# Autodesk Inventor assembly: 途中
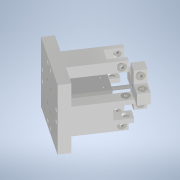
[picture p0: Inventor's stored thumbnail of the model, 180x180]
Saved by Autodesk Inventor 2021 (Build 250183000, 183)
## iProperties
Created: 2021-10-17
Part Number: 途中
Document SubType Name: Assembly
Designer: ryusei
Author: ryusei
## Documents named in this file (9)
- C:\Users\ryusei\Documents\Inventor\robot_design3\完成版\途中.iam
- C:\Users\ryusei\Documents\Inventor\robot_design3\試作品2号\部品\土台.ipt
- C:\Users\ryusei\Documents\Inventor\robot_design3\試作品2号\部品\アーム支え.ipt
- C:\Users\ryusei\Documents\Inventor\robot_design3\試作品2号\部品\シリンダ固定.ipt
- C:\Users\ryusei\Documents\Inventor\robot_design3\試作品2号\部品\MBDA6×15_シリンダコガネイ\本体.ipt
- C:\Users\ryusei\Documents\Inventor\robot_design3\試作品2号\部品\MBDA6×15_シリンダコガネイ\伸びるやつ１.ipt
- C:\Users\ryusei\Documents\Inventor\robot_design3\試作品2号\部品\MBDA6×15_シリンダコガネイ\伸びるやつ2.ipt
- C:\Users\ryusei\Documents\Inventor\robot_design3\試作品2号\部品\シリンダ先端パーツ.ipt
- C:\Users\ryusei\Documents\Inventor\robot_design3\試作品2号\部品\MF63ZZ_ベアリング.ipt
## Components (27 placed, 8 different names)
1. 土台:1
2. アーム支え:1
3. アーム支え:2
4. アーム支え:3
5. アーム支え:4
6. シリンダ固定:1
7. シリンダ固定:2
8. 本体:1
9. 伸びるやつ１:1
10. 伸びるやつ2:1
11. シリンダ先端パーツ:1 — 挿入:34
12. MF63ZZ_ベアリング:1
13. MF63ZZ_ベアリング:2
14. MF63ZZ_ベアリング:3
15. MF63ZZ_ベアリング:4
16. MF63ZZ_ベアリング:5
17. MF63ZZ_ベアリング:6
18. MF63ZZ_ベアリング:7
19. MF63ZZ_ベアリング:8
20. MF63ZZ_ベアリング:9
21. MF63ZZ_ベアリング:10
22. MF63ZZ_ベアリング:11 — 挿入:34
23. MF63ZZ_ベアリング:12
24. MF63ZZ_ベアリング:13
25. MF63ZZ_ベアリング:14
26. MF63ZZ_ベアリング:15
27. MF63ZZ_ベアリング:16
## Relationships (37: Insert 34, Mate 1, CylindricalJoint 1, Angle 1)
- [Insert]: 土台:1 ↔ アーム支え:1
- [Insert]: 土台:1 ↔ アーム支え:1
- [Insert]: 土台:1 ↔ アーム支え:2
- [Insert]: 土台:1 ↔ アーム支え:2
- [Insert]: 土台:1 ↔ アーム支え:3
- [Insert]: 土台:1 ↔ アーム支え:3
- [Insert]: 土台:1 ↔ アーム支え:4
- [Insert]: 土台:1 ↔ アーム支え:4
- [Insert]: 土台:1 ↔ シリンダ固定:2
- [Insert]: 土台:1 ↔ シリンダ固定:2
- [Insert]: 土台:1 ↔ シリンダ固定:1
- [Insert]: 土台:1 ↔ シリンダ固定:1
- [Insert]: シリンダ固定:1 ↔ 本体:1
- [Insert]: シリンダ固定:1 ↔ 本体:1
- [Insert]: シリンダ固定:2 ↔ 本体:1
- [Insert]: シリンダ固定:2 ↔ 本体:1
- [Insert]: 伸びるやつ１:1 ↔ 伸びるやつ2:1
- [Mate]: 本体:1 ↔ 伸びるやつ１:1
- [CylindricalJoint]: 本体:1 ↔ 伸びるやつ１:1
- [Insert]: 伸びるやつ2:1 ↔ シリンダ先端パーツ:1
- [Angle] (0 deg): アーム支え:4 ↔ シリンダ先端パーツ:1
- [Insert]: アーム支え:2 ↔ MF63ZZ_ベアリング:5
- [Insert]: アーム支え:2 ↔ MF63ZZ_ベアリング:16
- [Insert]: アーム支え:1 ↔ MF63ZZ_ベアリング:1
- [Insert]: アーム支え:1 ↔ MF63ZZ_ベアリング:3
- [Insert]: アーム支え:4 ↔ MF63ZZ_ベアリング:2
- [Insert]: アーム支え:4 ↔ MF63ZZ_ベアリング:7
- [Insert]: アーム支え:3 ↔ MF63ZZ_ベアリング:9
- [Insert]: アーム支え:3 ↔ MF63ZZ_ベアリング:15
- [Insert]: シリンダ先端パーツ:1 ↔ MF63ZZ_ベアリング:4
- [Insert]: シリンダ先端パーツ:1 ↔ MF63ZZ_ベアリング:6
- [Insert]: シリンダ先端パーツ:1 ↔ MF63ZZ_ベアリング:14
- [Insert]: シリンダ先端パーツ:1 ↔ MF63ZZ_ベアリング:8
- [Insert]: シリンダ先端パーツ:1 ↔ MF63ZZ_ベアリング:13
- [Insert]: シリンダ先端パーツ:1 ↔ MF63ZZ_ベアリング:10
- [Insert]: シリンダ先端パーツ:1 ↔ MF63ZZ_ベアリング:12
- 挿入:34 [Insert]: シリンダ先端パーツ:1 ↔ MF63ZZ_ベアリング:11
## Named parameters: d0_d29 = 0 mm, d1_d30 = 0 mm, d2_d31 = 0 mm, d3_d32 = 0 mm, d4_d33 = 0 mm, d5_d34 = 0 mm, d6_d35 = 0 mm, d7_d36 = 0 mm, d8_d37 = 0 mm, d9_d38 = 0 mm, d16_d23 = 0 deg, d17_d26 = 0 mm, d18_d27 = 0 mm, d19_d28 = 0 mm
